# Autodesk Inventor assembly: wing
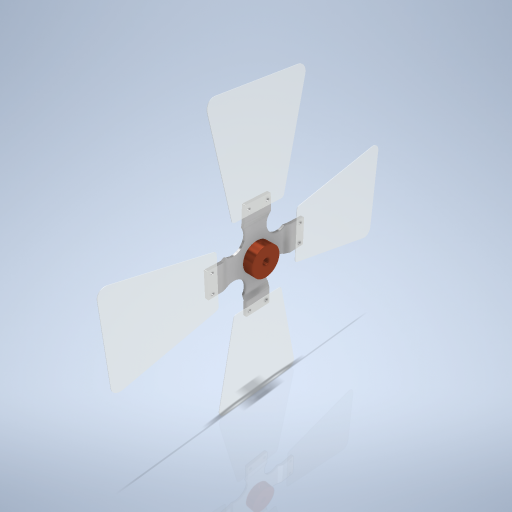
[picture p0: Inventor's stored thumbnail of the model, 512x512]
Saved by Autodesk Inventor 2024.2 (Build 282272000, 272)
## iProperties
Created: 2024-05-16
Part Number: wing
Document SubType Name: Assembly
Designer: Fabri
Author: Fabri
## Documents named in this file (3)
- C:\Users\Fabri\Documents\Inventor\Stirlingfan\wing.iam
- C:\Users\Fabri\Documents\Inventor\Stirlingfan\Propeller_complete.iam
- C:\Users\Fabri\Documents\Inventor\Stirlingfan\30.ipt
## Components (2 placed, 2 different names)
1. Propeller_complete:1 [sub-assembly] — Einfügen:1
2. 30:1 — Einfügen:1
## Relationships (1: Insert 1)
- Einfügen:1 [Insert]: Propeller_complete:1 ↔ 30:1
